# Autodesk Inventor assembly: one_unit
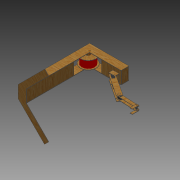
[picture p0: Inventor's stored thumbnail of the model, 180x180]
Saved by Autodesk Inventor 2013 (Build 170138000, 138)
## iProperties
Created: 2014-10-20
Part Number: one_unit
Document SubType Name: Assembly
Designer: Masta
Author: Masta
## Documents named in this file (5)
- D:\DrOctopus\3D model\one_unit.iam
- D:\DrOctopus\3D model\stand\stand.iam
- D:\DrOctopus\3D model\arm\arm.iam
- D:\DrOctopus\3D model\filament.ipt
- D:\DrOctopus\3D model\roll.ipt
## Components (4 placed, 4 different names)
1. stand:1 [sub-assembly] — Insert:1, Angle:1, Tangent:1, Mate:1
2. arm:1 [sub-assembly] — Insert:1, Angle:1
3. filament:1 — Insert:2
4. roll:1 — Insert:2, Tangent:1, Mate:1
## Relationships (5: Insert 2, Angle 1, Tangent 1, Mate 1)
- Insert:1: stand:1 ↔ arm:1
- Angle:1 (0 deg): stand:1 ↔ arm:1
- Insert:2: filament:1 ↔ roll:1
- Tangent:1: stand:1 ↔ roll:1
- Mate:1 (20 mm): stand:1 ↔ roll:1
